# Autodesk Inventor assembly: base plate
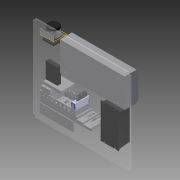
[picture p0: Inventor's stored thumbnail of the model, 180x180]
Saved by Autodesk Inventor 2012 (Build 160160000, 160)
## iProperties
Created: 2012-05-12
Part Number: base plate
Document SubType Name: Assembly
Designer: esv
Author: esv
## Documents named in this file (10)
- C:\Users\esv\masters\CAD\base plate.iam
- C:\Users\esv\masters\CAD\cRIO\Inventor\cRIO with Modules.iam
- C:\Users\esv\masters\CAD\Cap\Cap.ipt
- C:\Users\esv\masters\CAD\Frame\base plate.ipt
- C:\Users\esv\masters\CAD\cRIO\cRIO Breakout Keepout.ipt
- C:\Users\esv\masters\CAD\13.8V Supply\supply-13.8.ipt
- C:\Users\esv\masters\CAD\Sabertooth\sabertooth keepout.ipt
- C:\Users\esv\masters\CAD\Inverter\inverter.ipt
- C:\Users\esv\masters\CAD\cRIO\cRIO bracket.ipt
- C:\Users\esv\masters\CAD\Relay\relay.ipt
## Components (9 placed, 9 different names)
1. cRIO with Modules:1 [sub-assembly] — Mate:1, Flush:1, Flush:2, Insert:6, Insert:7
2. Cap:1 — Tangent:1, Flush:3, Tangent:2
3. base plate:1 — Insert:1, Insert:2, Insert:3, Angle:1, Insert:4, Insert:5, Insert:8, Insert:9, Insert:10, Angle:2
4. cRIO Breakout Keepout:1 — Mate:1, Flush:1, Flush:2
5. supply-13.8:1 — Insert:3, Angle:1
6. sabertooth keepout:1 — Insert:4, Insert:5
7. inverter:1 — Insert:1, Insert:2
8. cRIO bracket:1 — Insert:6, Insert:7, Insert:8, Insert:9, Tangent:1, Flush:3, Tangent:2
9. relay:1 — Insert:10, Angle:2
## Relationships (18: Insert 10, Flush 3, Angle 2, Tangent 2, Mate 1)
- Insert:1: base plate:1 ↔ inverter:1
- Insert:2: base plate:1 ↔ inverter:1
- Mate:1: cRIO with Modules:1 ↔ cRIO Breakout Keepout:1
- Flush:1: cRIO with Modules:1 ↔ cRIO Breakout Keepout:1
- Flush:2: cRIO with Modules:1 ↔ cRIO Breakout Keepout:1
- Insert:3: base plate:1 ↔ supply-13.8:1
- Angle:1 (0 deg): base plate:1 ↔ supply-13.8:1
- Insert:4: base plate:1 ↔ sabertooth keepout:1
- Insert:5: base plate:1 ↔ sabertooth keepout:1
- Insert:6: cRIO with Modules:1 ↔ cRIO bracket:1
- Insert:7: cRIO with Modules:1 ↔ cRIO bracket:1
- Insert:8: base plate:1 ↔ cRIO bracket:1
- Insert:9: base plate:1 ↔ cRIO bracket:1
- Tangent:1: Cap:1 ↔ cRIO bracket:1
- Flush:3 (50.8 mm): Cap:1 ↔ cRIO bracket:1
- Tangent:2: Cap:1 ↔ cRIO bracket:1
- Insert:10: base plate:1 ↔ relay:1
- Angle:2 (0 deg): base plate:1 ↔ relay:1
